# Autodesk Inventor assembly: Enclosure
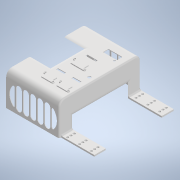
[picture p0: Inventor's stored thumbnail of the model, 180x180]
Saved by Autodesk Inventor 2020 (Build 240168000, 168)
## iProperties
Created: 2020-02-13
Part Number: Enclosure
Document SubType Name: Assembly
Designer: pp445
Author: pp445
## Documents named in this file (4)
- D:\MENG Project\Open-AMR-Hardware\Hardware\MCAD\Enclosure.iam
- D:\MENG Project\Open-AMR-Hardware\Hardware\MCAD\CustomParts\Enclosure.ipt
- D:\MENG Project\Open-AMR-Hardware\Hardware\MCAD\CustomParts\USB Mount.ipt
- D:\MENG Project\Open-AMR-Hardware\Hardware\MCAD\CustomParts\HDMI Mount.ipt
## Components (4 placed, 3 different names)
1. Enclosure:1 — Flush:1, Flush:2, Flush:3, Mate:1, Mate:2, Mate:3, Mate:4, Mate:5, Mate:6, Mate:7, Mate:8, Mate:9
2. USB Mount:1 — Mate:2, Mate:3, Mate:4
3. USB Mount:2 — Mate:1, Mate:5, Mate:6
4. HDMI Mount:1 — Mate:7, Mate:8, Mate:9
## Relationships (12: Mate 9, Flush 3)
- Flush:1: Enclosure:1
- Flush:2: Enclosure:1
- Flush:3: Enclosure:1
- Mate:1: Enclosure:1 ↔ USB Mount:2
- Mate:2: Enclosure:1 ↔ USB Mount:1
- Mate:3: Enclosure:1 ↔ USB Mount:1
- Mate:4: Enclosure:1 ↔ USB Mount:1
- Mate:5: Enclosure:1 ↔ USB Mount:2
- Mate:6: Enclosure:1 ↔ USB Mount:2
- Mate:7: Enclosure:1 ↔ HDMI Mount:1
- Mate:8: Enclosure:1 ↔ HDMI Mount:1
- Mate:9: Enclosure:1 ↔ HDMI Mount:1
